# Autodesk Inventor assembly: xnucleo
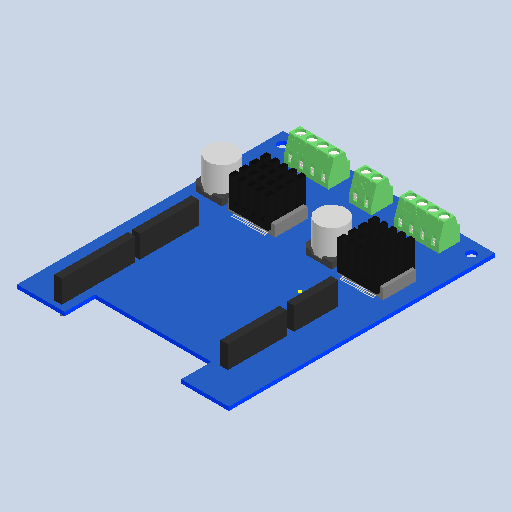
[picture p0: Inventor's stored thumbnail of the model, 512x512]
Saved by Autodesk Inventor 2023 (Build 270158000, 158)
## iProperties
Created: 2023-11-04
Part Number: xnucleo
Document SubType Name: Assembly
Designer: eleves
Author: eleves
## Documents named in this file (7)
- C:\Users\eleves\Desktop\export\blocdriver\xnucleo\xnucleo.iam
- C:\Users\eleves\Desktop\export\blocdriver\xnucleo\xucleobase.ipt
- C:\Users\eleves\Desktop\export\blocdriver\xnucleo\SOIC_470PD_STM.ipt
- C:\Users\eleves\Desktop\export\blocdriver\xnucleo\PCAP_10x10-ELECT_NCA.ipt
- C:\Users\eleves\Desktop\export\blocdriver\xnucleo\Heatsink_13x13x10.ipt
- C:\Users\eleves\Desktop\export\blocdriver\conn2\1727010.iam
- C:\Users\eleves\Desktop\export\blocdriver\conn4\1727036.iam
## Components (10 placed, 6 different names)
1. xucleobase:1 — Placage:1, Angle:1, Placage:2, Placage:3, Placage:4, Placage:7, Angle:2, Placage:8, Angle:3, Placage:9
2. SOIC_470PD_STM:1 — Placage:1, Angle:1, Placage:6
3. SOIC_470PD_STM:2 — Placage:3, Placage:5
4. PCAP_10x10-ELECT_NCA:1 — Placage:2
5. PCAP_10x10-ELECT_NCA:2 — Placage:4
6. Heatsink_13x13x10:1 — Placage:5
7. Heatsink_13x13x10:2 — Placage:6
8. 1727010:1 [sub-assembly] — Placage:7, Angle:2
9. 1727036:1 [sub-assembly] — Placage:8, Angle:3
10. 1727036:2 [sub-assembly] — Placage:9
## Relationships (12: Mate 9, Angle 3)
- Placage:1 [Mate]: xucleobase:1 ↔ SOIC_470PD_STM:1
- Angle:1 (180 deg): xucleobase:1 ↔ SOIC_470PD_STM:1
- Placage:2 [Mate]: xucleobase:1 ↔ PCAP_10x10-ELECT_NCA:1
- Placage:3 [Mate]: xucleobase:1 ↔ SOIC_470PD_STM:2
- Placage:4 [Mate]: xucleobase:1 ↔ PCAP_10x10-ELECT_NCA:2
- Placage:5 [Mate] (-2 mm): SOIC_470PD_STM:2 ↔ Heatsink_13x13x10:1
- Placage:6 [Mate] (-2 mm): SOIC_470PD_STM:1 ↔ Heatsink_13x13x10:2
- Placage:7 [Mate]: xucleobase:1 ↔ 1727010:1
- Angle:2 (0 deg): xucleobase:1 ↔ 1727010:1
- Placage:8 [Mate]: xucleobase:1 ↔ 1727036:1
- Angle:3 (0 deg): xucleobase:1 ↔ 1727036:1
- Placage:9 [Mate]: xucleobase:1 ↔ 1727036:2
